# Autodesk Inventor assembly: WheelIntake4.0
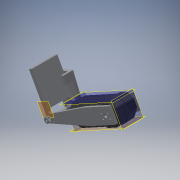
[picture p0: Inventor's stored thumbnail of the model, 180x180]
Saved by Autodesk Inventor 2017 (Build 210142000, 142)
## iProperties
Created: 2017-12-13
Part Number: WheelIntake4.0
Document SubType Name: Assembly
Designer: User
Author: User
## Documents named in this file (5)
- C:\Robotics\CAD\2017-18_CAD\WheelIntake4.0.iam
- C:\Robotics\CAD\COTSParts\Rev\REV-41-1300.ipt
- C:\Robotics\CAD\2017-18_CAD\WheelIntakeMount4.0.ipt
- C:\Robotics\CAD\COTSParts\Fasteners\97345A171_TYPE 316 STAINLESS STEEL SHOULDER SCREW.ipt
- C:\Robotics\CAD\2017-18_CAD\WheelIntake4.0Base.ipt
## Components (4 placed, 4 different names)
1. REV-41-1300:1 — Insert:1, Insert:2
2. WheelIntakeMount4.0:1 — Insert:1, Insert:2, Insert:3
3. 97345A171_TYPE 316 STAINLESS STEEL SHOULDER SCREW:1 — Insert:3, Insert:4
4. WheelIntake4.0Base:1 — Insert:4
## Relationships (4: Insert 4)
- Insert:1: REV-41-1300:1 ↔ WheelIntakeMount4.0:1
- Insert:2: REV-41-1300:1 ↔ WheelIntakeMount4.0:1
- Insert:3: WheelIntakeMount4.0:1 ↔ 97345A171_TYPE 316 STAINLESS STEEL SHOULDER SCREW:1
- Insert:4: 97345A171_TYPE 316 STAINLESS STEEL SHOULDER SCREW:1 ↔ WheelIntake4.0Base:1
